# Autodesk Inventor assembly: MARCO CORREDERA 1400X1200 MM
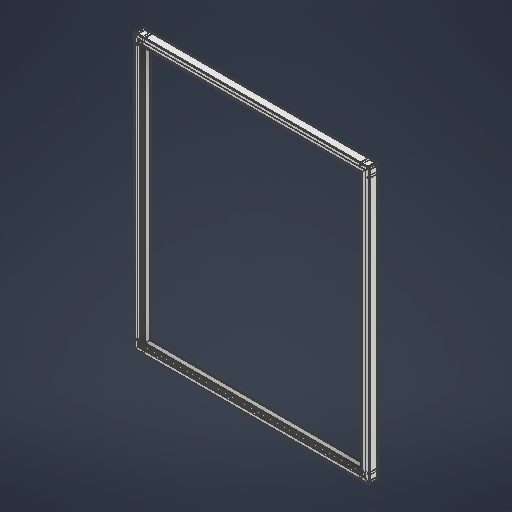
[picture p0: Inventor's stored thumbnail of the model, 512x512]
Saved by Autodesk Inventor 2025 (Build 290162000, 162)
## iProperties
Created: 2026-02-13
Part Number: MARCO CORREDERA 1400X1200 MM
Document SubType Name: Assembly
Designer: Frank
Author: Frank
## Documents named in this file (10)
- C:\Users\rolan\OneDrive\Documentos\Inventor\Projects\CARPINTERIA ALUMINIO\PUERTAS Y VENTANAS\VENTANAS\MARCO DE CORREDERA\MARCO CORREDERA SP40-09 EXT 1400x1200.iam
- MARCO CORREDERA SP40-09 EXT 1400x1200.iam
- C:\Users\rolan\OneDrive\Documentos\Inventor\Projects\CARPINTERIA ALUMINIO\PUERTAS Y VENTANAS\VENTANAS\MARCO DE CORREDERA\SP40-09 MARCO CORREDERA 1400 MM.ipt
- C:\Users\rolan\OneDrive\Documentos\Inventor\Projects\CARPINTERIA ALUMINIO\PUERTAS Y VENTANAS\VENTANAS\MARCO DE CORREDERA\SP40-09 MARCO CORREDERA 1200 MM.ipt
- C:\Users\rolan\OneDrive\Documentos\Inventor\Projects\CARPINTERIA ALUMINIO\PUERTAS Y VENTANAS\VENTANAS\MARCO DE CORREDERA\BRA-13 ESCUADRA UNIÓN 45 37 mm.ipt
- C:\Users\rolan\OneDrive\Documentos\Inventor\Projects\CARPINTERIA ALUMINIO\PUERTAS Y VENTANAS\VENTANAS\MARCO DE CORREDERA\SP40-09 MARCO CORREDERA 1200 MM_MIR.ipt
- C:\Users\rolan\OneDrive\Documentos\Inventor\Projects\CARPINTERIA ALUMINIO\PUERTAS Y VENTANAS\VENTANAS\MARCO DE CORREDERA\BRA-13 ESCUADRA UNIÓN 45 37 mm_MIR.ipt
- C:\Users\rolan\OneDrive\Documentos\Inventor\Projects\CARPINTERIA ALUMINIO\PUERTAS Y VENTANAS\VENTANAS\MARCO DE CORREDERA\SP40-09 MARCO CORREDERA 1400 MM_MIR.ipt
- C:\Users\rolan\OneDrive\Documentos\Inventor\Projects\CARPINTERIA ALUMINIO\PUERTAS Y VENTANAS\VENTANAS\MARCO DE CORREDERA\BRA-13 ESCUADRA UNIÓN 45 37 mm_MIR1.ipt
- C:\Users\rolan\OneDrive\Documentos\Inventor\Projects\CARPINTERIA ALUMINIO\PUERTAS Y VENTANAS\VENTANAS\MARCO DE CORREDERA\BRA-13 ESCUADRA UNIÓN 45 37 mm_MIR2.ipt
## Components (8 placed, 8 different names)
1. SP40-09 MARCO CORREDERA 1400 MM:1 — Coincidencia:1, Coincidencia:2, Coincidencia:4, Nivelación:1, Coincidencia:11, Coincidencia:12, Nivelación:2, Coincidencia:16
2. SP40-09 MARCO CORREDERA 1200 MM:1 — Coincidencia:3, Coincidencia:4, Coincidencia:8, Coincidencia:9, Coincidencia:10, Nivelación:1, Coincidencia:17
3. BRA-13 ESCUADRA UNIÓN 45 37 mm:1 — Coincidencia:1, Coincidencia:2, Coincidencia:3
4. SP40-09 MARCO CORREDERA 1200 MM_MIR:1 — Coincidencia:5, Coincidencia:12, Nivelación:2, Coincidencia:13, Coincidencia:14
5. BRA-13 ESCUADRA UNIÓN 45 37 mm_MIR:1 — Coincidencia:5, Coincidencia:11, Coincidencia:16
6. SP40-09 MARCO CORREDERA 1400 MM_MIR:1 — Coincidencia:6, Coincidencia:7, Coincidencia:8, Coincidencia:10, Coincidencia:15, Coincidencia:18
7. BRA-13 ESCUADRA UNIÓN 45 37 mm_MIR1:1 — Coincidencia:6, Coincidencia:7, Coincidencia:9
8. BRA-13 ESCUADRA UNIÓN 45 37 mm_MIR2:1 — Coincidencia:13, Coincidencia:14, Coincidencia:15
## Relationships (20: Mate 18, Flush 2)
- Coincidencia:1 [Mate]: SP40-09 MARCO CORREDERA 1400 MM:1 ↔ BRA-13 ESCUADRA UNIÓN 45 37 mm:1
- Coincidencia:2 [Mate] (1 mm): SP40-09 MARCO CORREDERA 1400 MM:1 ↔ BRA-13 ESCUADRA UNIÓN 45 37 mm:1
- Coincidencia:3 [Mate]: SP40-09 MARCO CORREDERA 1200 MM:1 ↔ BRA-13 ESCUADRA UNIÓN 45 37 mm:1
- Coincidencia:4 [Mate]: SP40-09 MARCO CORREDERA 1400 MM:1 ↔ SP40-09 MARCO CORREDERA 1200 MM:1
- Coincidencia:5 [Mate]: SP40-09 MARCO CORREDERA 1200 MM_MIR:1 ↔ BRA-13 ESCUADRA UNIÓN 45 37 mm_MIR:1
- Coincidencia:6 [Mate] (1 mm): SP40-09 MARCO CORREDERA 1400 MM_MIR:1 ↔ BRA-13 ESCUADRA UNIÓN 45 37 mm_MIR1:1
- Coincidencia:7 [Mate]: SP40-09 MARCO CORREDERA 1400 MM_MIR:1 ↔ BRA-13 ESCUADRA UNIÓN 45 37 mm_MIR1:1
- Coincidencia:8 [Mate]: SP40-09 MARCO CORREDERA 1200 MM:1 ↔ SP40-09 MARCO CORREDERA 1400 MM_MIR:1
- Coincidencia:9 [Mate]: SP40-09 MARCO CORREDERA 1200 MM:1 ↔ BRA-13 ESCUADRA UNIÓN 45 37 mm_MIR1:1
- Coincidencia:10 [Mate]: SP40-09 MARCO CORREDERA 1200 MM:1 ↔ SP40-09 MARCO CORREDERA 1400 MM_MIR:1
- Nivelación:1 [Flush]: SP40-09 MARCO CORREDERA 1400 MM:1 ↔ SP40-09 MARCO CORREDERA 1200 MM:1
- Coincidencia:11 [Mate]: SP40-09 MARCO CORREDERA 1400 MM:1 ↔ BRA-13 ESCUADRA UNIÓN 45 37 mm_MIR:1
- Coincidencia:12 [Mate]: SP40-09 MARCO CORREDERA 1400 MM:1 ↔ SP40-09 MARCO CORREDERA 1200 MM_MIR:1
- Nivelación:2 [Flush]: SP40-09 MARCO CORREDERA 1400 MM:1 ↔ SP40-09 MARCO CORREDERA 1200 MM_MIR:1
- Coincidencia:13 [Mate]: SP40-09 MARCO CORREDERA 1200 MM_MIR:1 ↔ BRA-13 ESCUADRA UNIÓN 45 37 mm_MIR2:1
- Coincidencia:14 [Mate] (1 mm): SP40-09 MARCO CORREDERA 1200 MM_MIR:1 ↔ BRA-13 ESCUADRA UNIÓN 45 37 mm_MIR2:1
- Coincidencia:15 [Mate]: SP40-09 MARCO CORREDERA 1400 MM_MIR:1 ↔ BRA-13 ESCUADRA UNIÓN 45 37 mm_MIR2:1
- Coincidencia:16 [Mate] (1 mm): SP40-09 MARCO CORREDERA 1400 MM:1 ↔ BRA-13 ESCUADRA UNIÓN 45 37 mm_MIR:1
- Coincidencia:17 [Mate]: SP40-09 MARCO CORREDERA 1200 MM:1
- Coincidencia:18 [Mate]: SP40-09 MARCO CORREDERA 1400 MM_MIR:1
